# Autodesk Inventor assembly: Ensamblaje1
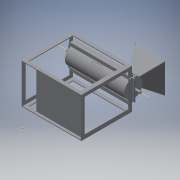
[picture p0: Inventor's stored thumbnail of the model, 180x180]
Saved by Autodesk Inventor 2019 (Build 230136000, 136)
## iProperties
Created: 2021-07-03
Part Number: Ensamblaje1
Material: Genérico
Document SubType Name: Assembly
Designer: Usuario
Author: Usuario
## Documents named in this file (5)
- C:\Users\DanielAlvaradoPelaez\Desktop\Espol S6\comunitarias\diseño\Ensamblaje1.iam
- C:\Users\DanielAlvaradoPelaez\Desktop\Espol S6\comunitarias\diseño\mesa.ipt
- C:\Users\DanielAlvaradoPelaez\Desktop\Espol S6\comunitarias\diseño\cilindro exterior.ipt
- C:\Users\DanielAlvaradoPelaez\Desktop\Espol S6\comunitarias\diseño\cernidera.ipt
- C:\Users\DanielAlvaradoPelaez\Desktop\Espol S6\comunitarias\diseño\eje de moler.ipt
## Components (4 placed, 4 different names)
1. mesa:1 — Coincidencia:3, Coincidencia:4, Coincidencia:5
2. cilindro exterior:1 — Coincidencia:1, Coincidencia:2, Coincidencia:3, Coincidencia:4, Coincidencia:5, Nivelación:1, Coincidencia:6, Coincidencia:7
3. cernidera:1 — Coincidencia:1, Coincidencia:2, Nivelación:1
4. eje de moler:1 — Coincidencia:6, Coincidencia:7
## Relationships (8: Mate 7, Flush 1)
- Coincidencia:1 [Mate]: cilindro exterior:1 ↔ cernidera:1
- Coincidencia:2 [Mate]: cilindro exterior:1 ↔ cernidera:1
- Coincidencia:3 [Mate]: mesa:1 ↔ cilindro exterior:1
- Coincidencia:4 [Mate]: mesa:1 ↔ cilindro exterior:1
- Coincidencia:5 [Mate]: mesa:1 ↔ cilindro exterior:1
- Nivelación:1 [Flush] (197.5 mm): cilindro exterior:1 ↔ cernidera:1
- Coincidencia:6 [Mate]: cilindro exterior:1 ↔ eje de moler:1
- Coincidencia:7 [Mate]: cilindro exterior:1 ↔ eje de moler:1
